# Autodesk Inventor assembly: HexapodShelled
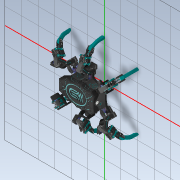
[picture p0: Inventor's stored thumbnail of the model, 180x180]
Saved by Autodesk Inventor 2020 (Build 240168000, 168)
## iProperties
Created: 2020-02-19
Part Number: HexapodShelled
Document SubType Name: Assembly
Designer: Turing
Author: Turing
## Documents named in this file (20)
- D:\Hexapod Final Fucking Version\HexapodShelled.iam
- D:\Hexapod Final Fucking Version\BodyMid.ipt
- D:\Hexapod Final Fucking Version\BodyBotSup.ipt
- D:\Hexapod Final Fucking Version\Power Button.ipt
- D:\Hexapod Final Fucking Version\LegDemoRight.iam
- D:\Hexapod Final Fucking Version\PCBSupport.iam
- D:\Hexapod Final Fucking Version\BodyCasing.iam
- D:\Hexapod Final Fucking Version\BodyBot.iam
- D:\Hexapod Final Fucking Version\Bearing1.iam
- D:\Hexapod Final Fucking Version\Bearing2.iam
- D:\Hexapod Final Fucking Version\Bearing3.iam
- D:\Hexapod Final Fucking Version\Bearing4.iam
- D:\Hexapod Final Fucking Version\Bearing5.iam
- D:\Hexapod Final Fucking Version\Bearing6.iam
- D:\Hexapod Final Fucking Version\XL4016E1 8A Buck Converter.ipt
- D:\Hexapod Final Fucking Version\LegDemoRightLeft1.iam
- D:\Hexapod Final Fucking Version\HexapodShelled\Design Accelerator\Bolted Connection1.iam
- D:\Hexapod Final Fucking Version\HexapodShelled\Design Accelerator\Bolted Connection3.iam
- D:\Hexapod Final Fucking Version\HexapodShelled\Design Accelerator\Bolted Connection4.iam
- D:\Hexapod Final Fucking Version\HexapodShelled\Design Accelerator\Bolted Connection5.iam
## Components (23 placed, 11 different names)
1. BodyMid:1 — Rigid:31, Rigid:32, Mate:9, Mate:10
2. Power Button:1 — Rigid:31
3. PCBSupport:1 [sub-assembly] — Rigid:37, Mate:15, Mate:16
4. BodyCasing:1 [sub-assembly] — Rigid:39
5. BodyBotSup:1 — Rigid:36
6. BodyBot:1 [sub-assembly] — Rigid:32, Rigid:36, Rigid:37, Rigid:39, Rigid:43, Rigid:44, Rigid:45, Rigid:46, Mate:7, Flush:7, Mate:8, Flush:8, Rigid:47, Rigid:48, Rigid:49
7. LegDemoRight:1 [sub-assembly] — Rigid:43
8. LegDemoRight:2 [sub-assembly] — Rigid:44
9. LegDemoRight:3 [sub-assembly] — Rigid:45
10. Body_Bearing:1 [sub-assembly]
11. Body_Bearing:2 [sub-assembly]
12. Body_Bearing:3 [sub-assembly]
13. Body_Bearing:4 [sub-assembly] — Mate:7, Flush:7
14. Body_Bearing:5 [sub-assembly] — Mate:8, Flush:8
15. Body_Bearing:6 [sub-assembly]
16. XL4016E1 8A Buck Converter:1 — Rigid:46, Mate:11, Mate:12, Mate:13, Mate:14
17. LegDemoRightLeft:1 [sub-assembly] — Rigid:47
18. LegDemoRightLeft:2 [sub-assembly] — Rigid:48
19. LegDemoRightLeft:3 [sub-assembly] — Rigid:49
20. Body Bolted Connection:1 [sub-assembly] — Mate:9, Mate:10
21. Body Bolted Connection:2 [sub-assembly] — Mate:11, Mate:12
22. Body Bolted Connection:3 [sub-assembly] — Mate:13, Mate:14
23. Body Bolted Connection:4 [sub-assembly] — Mate:15, Mate:16
## Relationships (24: WeldJoint 12, Mate 10, Flush 2)
- Rigid:31 [WeldJoint]: BodyMid:1 ↔ Power Button:1
- Rigid:32 [WeldJoint]: BodyMid:1 ↔ BodyBot:1
- Rigid:36 [WeldJoint]: BodyBotSup:1 ↔ BodyBot:1
- Rigid:37 [WeldJoint]: PCBSupport:1 ↔ BodyBot:1
- Rigid:39 [WeldJoint]: BodyCasing:1 ↔ BodyBot:1
- Rigid:43 [WeldJoint]: BodyBot:1 ↔ LegDemoRight:1
- Rigid:44 [WeldJoint]: BodyBot:1 ↔ LegDemoRight:2
- Rigid:45 [WeldJoint]: BodyBot:1 ↔ LegDemoRight:3
- Rigid:46 [WeldJoint]: BodyBot:1 ↔ XL4016E1 8A Buck Converter:1
- Mate:7: BodyBot:1 ↔ Body_Bearing:4
- Flush:7: BodyBot:1 ↔ Body_Bearing:4
- Mate:8: BodyBot:1 ↔ Body_Bearing:5
- Flush:8: BodyBot:1 ↔ Body_Bearing:5
- Rigid:47 [WeldJoint]: BodyBot:1 ↔ LegDemoRightLeft:1
- Rigid:48 [WeldJoint]: BodyBot:1 ↔ LegDemoRightLeft:2
- Rigid:49 [WeldJoint]: BodyBot:1 ↔ LegDemoRightLeft:3
- Mate:9: BodyMid:1 ↔ Body Bolted Connection:1
- Mate:10: BodyMid:1 ↔ Body Bolted Connection:1
- Mate:11: XL4016E1 8A Buck Converter:1 ↔ Body Bolted Connection:2
- Mate:12: XL4016E1 8A Buck Converter:1 ↔ Body Bolted Connection:2
- Mate:13: XL4016E1 8A Buck Converter:1 ↔ Body Bolted Connection:3
- Mate:14: XL4016E1 8A Buck Converter:1 ↔ Body Bolted Connection:3
- Mate:15: PCBSupport:1 ↔ Body Bolted Connection:4
- Mate:16: PCBSupport:1 ↔ Body Bolted Connection:4
